# Autodesk Inventor assembly: Base
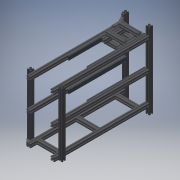
[picture p0: Inventor's stored thumbnail of the model, 180x180]
Saved by Autodesk Inventor 2016 (Build 200138000, 138)
## iProperties
Created: 2016-11-24
Part Number: Base
Material: 一般
Document SubType Name: Assembly
Designer: Daisuke
Author: Daisuke
## Documents named in this file (10)
- C:\Users\Daisuke\Documents\GitHub\CAD\Tomoato2016\Base\Base.iam
- C:\Users\Daisuke\Documents\GitHub\CAD\Tomoato2016\Base\HFS6-3030-750.ipt
- C:\Users\Daisuke\Documents\GitHub\CAD\Tomoato2016\Base\HFS6-3030-600.ipt
- C:\Users\Daisuke\Documents\GitHub\CAD\Tomoato2016\Base\HBLTF6-C_.ipt
- C:\Users\Daisuke\Documents\GitHub\CAD\Tomoato2016\Base\HFS6-3030-159.ipt
- C:\Users\Daisuke\Documents\GitHub\CAD\Tomoato2016\Base\HFS6-3030-500.ipt
- C:\Users\Daisuke\Documents\GitHub\CAD\Tomoato2016\Base\HBLFSNE6_.ipt
- C:\Users\Daisuke\Documents\GitHub\CAD\Tomoato2016\Base\SSRN3618.iam
- C:\Users\Daisuke\Documents\GitHub\CAD\Tomoato2016\Base\HFS6-3030-200.ipt
- C:\Users\Daisuke\Documents\GitHub\CAD\Tomoato2016\Base\HFS6-3030-140.ipt
## Components (26 placed, 9 different names)
1. HFS6-3030-750:1 — メイト:8, フラッシュ:9, フラッシュ:10, フラッシュ:32, フラッシュ:33, メイト:22, メイト:23
2. HFS6-3030-750:2 — メイト:9, フラッシュ:11, フラッシュ:12, メイト:21, メイト:24
3. HFS6-3030-750:3 — メイト:10, フラッシュ:13, フラッシュ:14, メイト:11, フラッシュ:16, フラッシュ:18, メイト:13, フラッシュ:19, フラッシュ:20, メイト:14, フラッシュ:23, フラッシュ:24, メイト:18, フラッシュ:28, フラッシュ:29
4. HFS6-3030-750:4 — メイト:7, フラッシュ:7, フラッシュ:8, メイト:12, フラッシュ:15, フラッシュ:17, フラッシュ:21, フラッシュ:22, メイト:15, フラッシュ:25, メイト:16, フラッシュ:26, フラッシュ:27
5. HFS6-3030-750:5 — メイト:6, フラッシュ:5, フラッシュ:6, フラッシュ:30, メイト:19, メイト:25
6. HFS6-3030-750:6 — メイト:1, フラッシュ:1, メイト:3, メイト:4, フラッシュ:31, メイト:20, メイト:26
7. HFS6-3030-600:1 — メイト:8, フラッシュ:9, フラッシュ:10, メイト:9, フラッシュ:11, フラッシュ:12, メイト:10, フラッシュ:13, フラッシュ:14
8. HFS6-3030-600:2 — メイト:1, フラッシュ:1, メイト:2, フラッシュ:2, フラッシュ:3, メイト:5, フラッシュ:4, メイト:6, フラッシュ:5, フラッシュ:6, メイト:7, フラッシュ:7, フラッシュ:8
9. HBLTF6-C_:1 — メイト:2, フラッシュ:2, フラッシュ:3, メイト:3
10. HBLTF6-C_:2 — メイト:4, メイト:5, フラッシュ:4
11. HFS6-3030-159:1 — メイト:14, フラッシュ:23, フラッシュ:24
12. HFS6-3030-159:2 — メイト:11, メイト:12, フラッシュ:15, フラッシュ:16, フラッシュ:17, フラッシュ:18
13. HFS6-3030-159:3 — メイト:13, フラッシュ:19, フラッシュ:20, フラッシュ:21, フラッシュ:22
14. HFS6-3030-500:1 — メイト:18, フラッシュ:28, フラッシュ:29
15. HFS6-3030-500:2 — メイト:15, フラッシュ:25, メイト:17
16. HBLFSNE6_:1 — メイト:16, メイト:17, フラッシュ:26, フラッシュ:27
17. SSRN3618:1 [sub-assembly] — フラッシュ:32, メイト:21, メイト:24
18. SSRN3618:2 [sub-assembly] — フラッシュ:31, メイト:20, メイト:26, フラッシュ:35, メイト:29, メイト:30
19. SSRN3618:3 [sub-assembly] — フラッシュ:33, メイト:22, メイト:23, フラッシュ:34, メイト:27, メイト:28
20. SSRN3618:4 [sub-assembly] — フラッシュ:30, メイト:19, メイト:25
21. HFS6-3030-200:1 — フラッシュ:34, メイト:27, メイト:28, フラッシュ:38, メイト:32, メイト:33, フラッシュ:39, フラッシュ:40, メイト:35, フラッシュ:43, フラッシュ:44
22. HFS6-3030-200:2 — フラッシュ:35, メイト:29, メイト:30, メイト:31, フラッシュ:36, フラッシュ:37, メイト:34, フラッシュ:41, フラッシュ:42
23. HFS6-3030-140:1 — メイト:31, フラッシュ:36, フラッシュ:37, フラッシュ:38, メイト:32
24. HFS6-3030-140:2 — メイト:33, フラッシュ:39, フラッシュ:40
25. HFS6-3030-140:3 — メイト:35, フラッシュ:41, フラッシュ:42
26. HFS6-3030-140:4 — メイト:34, フラッシュ:43, フラッシュ:44
## Relationships (79: Flush 44, Mate 35)
- メイト:1 [Mate]: HFS6-3030-750:6 ↔ HFS6-3030-600:2
- フラッシュ:1 [Flush]: HFS6-3030-750:6 ↔ HFS6-3030-600:2
- メイト:2 [Mate]: HFS6-3030-600:2 ↔ HBLTF6-C_:1
- フラッシュ:2 [Flush]: HFS6-3030-600:2 ↔ HBLTF6-C_:1
- フラッシュ:3 [Flush] (-5 mm): HFS6-3030-600:2 ↔ HBLTF6-C_:1
- メイト:3 [Mate]: HFS6-3030-750:6 ↔ HBLTF6-C_:1
- メイト:4 [Mate]: HFS6-3030-750:6 ↔ HBLTF6-C_:2
- メイト:5 [Mate]: HFS6-3030-600:2 ↔ HBLTF6-C_:2
- フラッシュ:4 [Flush] (5 mm): HFS6-3030-600:2 ↔ HBLTF6-C_:2
- メイト:6 [Mate]: HFS6-3030-750:5 ↔ HFS6-3030-600:2
- フラッシュ:5 [Flush]: HFS6-3030-750:5 ↔ HFS6-3030-600:2
- フラッシュ:6 [Flush] (285 mm): HFS6-3030-750:5 ↔ HFS6-3030-600:2
- メイト:7 [Mate]: HFS6-3030-750:4 ↔ HFS6-3030-600:2
- フラッシュ:7 [Flush]: HFS6-3030-750:4 ↔ HFS6-3030-600:2
- フラッシュ:8 [Flush] (55 mm): HFS6-3030-750:4 ↔ HFS6-3030-600:2
- メイト:8 [Mate]: HFS6-3030-750:1 ↔ HFS6-3030-600:1
- フラッシュ:9 [Flush]: HFS6-3030-750:1 ↔ HFS6-3030-600:1
- フラッシュ:10 [Flush] (55 mm): HFS6-3030-750:1 ↔ HFS6-3030-600:1
- メイト:9 [Mate]: HFS6-3030-750:2 ↔ HFS6-3030-600:1
- フラッシュ:11 [Flush]: HFS6-3030-750:2 ↔ HFS6-3030-600:1
- フラッシュ:12 [Flush] (285 mm): HFS6-3030-750:2 ↔ HFS6-3030-600:1
- メイト:10 [Mate]: HFS6-3030-750:3 ↔ HFS6-3030-600:1
- フラッシュ:13 [Flush]: HFS6-3030-750:3 ↔ HFS6-3030-600:1
- フラッシュ:14 [Flush] (55 mm): HFS6-3030-750:3 ↔ HFS6-3030-600:1
- メイト:11 [Mate]: HFS6-3030-750:3 ↔ HFS6-3030-159:2
- メイト:12 [Mate]: HFS6-3030-750:4 ↔ HFS6-3030-159:2
- フラッシュ:15 [Flush]: HFS6-3030-750:4 ↔ HFS6-3030-159:2
- フラッシュ:16 [Flush]: HFS6-3030-750:3 ↔ HFS6-3030-159:2
- フラッシュ:17 [Flush] (51 mm): HFS6-3030-750:4 ↔ HFS6-3030-159:2
- フラッシュ:18 [Flush] (51 mm): HFS6-3030-750:3 ↔ HFS6-3030-159:2
- メイト:13 [Mate]: HFS6-3030-750:3 ↔ HFS6-3030-159:3
- フラッシュ:19 [Flush]: HFS6-3030-750:3 ↔ HFS6-3030-159:3
- フラッシュ:20 [Flush] (51 mm): HFS6-3030-750:3 ↔ HFS6-3030-159:3
- フラッシュ:21 [Flush]: HFS6-3030-750:4 ↔ HFS6-3030-159:3
- フラッシュ:22 [Flush] (51 mm): HFS6-3030-750:4 ↔ HFS6-3030-159:3
- メイト:14 [Mate]: HFS6-3030-750:3 ↔ HFS6-3030-159:1
- フラッシュ:23 [Flush]: HFS6-3030-750:3 ↔ HFS6-3030-159:1
- フラッシュ:24 [Flush] (360 mm): HFS6-3030-750:3 ↔ HFS6-3030-159:1
- メイト:15 [Mate]: HFS6-3030-750:4 ↔ HFS6-3030-500:2
- フラッシュ:25 [Flush]: HFS6-3030-750:4 ↔ HFS6-3030-500:2
- メイト:16 [Mate]: HFS6-3030-750:4 ↔ HBLFSNE6_:1
- メイト:17 [Mate]: HFS6-3030-500:2 ↔ HBLFSNE6_:1
- フラッシュ:26 [Flush]: HFS6-3030-750:4 ↔ HBLFSNE6_:1
- フラッシュ:27 [Flush] (5 mm): HFS6-3030-750:4 ↔ HBLFSNE6_:1
- メイト:18 [Mate]: HFS6-3030-750:3 ↔ HFS6-3030-500:1
- フラッシュ:28 [Flush]: HFS6-3030-750:3 ↔ HFS6-3030-500:1
- フラッシュ:29 [Flush] (-30 mm): HFS6-3030-750:3 ↔ HFS6-3030-500:1
- フラッシュ:30 [Flush]: HFS6-3030-750:5 ↔ SSRN3618:4
- メイト:19 [Mate]: HFS6-3030-750:5 ↔ SSRN3618:4
- フラッシュ:31 [Flush]: HFS6-3030-750:6 ↔ SSRN3618:2
- メイト:20 [Mate]: HFS6-3030-750:6 ↔ SSRN3618:2
- フラッシュ:32 [Flush]: HFS6-3030-750:1 ↔ SSRN3618:1
- メイト:21 [Mate]: HFS6-3030-750:2 ↔ SSRN3618:1
- フラッシュ:33 [Flush]: HFS6-3030-750:1 ↔ SSRN3618:3
- メイト:22 [Mate]: HFS6-3030-750:1 ↔ SSRN3618:3
- メイト:23 [Mate]: HFS6-3030-750:1 ↔ SSRN3618:3
- メイト:24 [Mate]: HFS6-3030-750:2 ↔ SSRN3618:1
- メイト:25 [Mate]: HFS6-3030-750:5 ↔ SSRN3618:4
- メイト:26 [Mate]: HFS6-3030-750:6 ↔ SSRN3618:2
- フラッシュ:34 [Flush]: SSRN3618:3 ↔ HFS6-3030-200:1
- メイト:27 [Mate]: SSRN3618:3 ↔ HFS6-3030-200:1
- メイト:28 [Mate]: SSRN3618:3 ↔ HFS6-3030-200:1
- フラッシュ:35 [Flush]: SSRN3618:2 ↔ HFS6-3030-200:2
- メイト:29 [Mate]: SSRN3618:2 ↔ HFS6-3030-200:2
- メイト:30 [Mate]: SSRN3618:2 ↔ HFS6-3030-200:2
- メイト:31 [Mate]: HFS6-3030-200:2 ↔ HFS6-3030-140:1
- フラッシュ:36 [Flush]: HFS6-3030-200:2 ↔ HFS6-3030-140:1
- フラッシュ:37 [Flush] (-30 mm): HFS6-3030-200:2 ↔ HFS6-3030-140:1
- フラッシュ:38 [Flush] (30 mm): HFS6-3030-200:1 ↔ HFS6-3030-140:1
- メイト:32 [Mate]: HFS6-3030-200:1 ↔ HFS6-3030-140:1
- メイト:33 [Mate]: HFS6-3030-200:1 ↔ HFS6-3030-140:2
- フラッシュ:39 [Flush]: HFS6-3030-200:1 ↔ HFS6-3030-140:2
- フラッシュ:40 [Flush] (30 mm): HFS6-3030-200:1 ↔ HFS6-3030-140:2
- メイト:34 [Mate]: HFS6-3030-200:2 ↔ HFS6-3030-140:4
- メイト:35 [Mate]: HFS6-3030-200:1 ↔ HFS6-3030-140:3
- フラッシュ:41 [Flush]: HFS6-3030-200:2 ↔ HFS6-3030-140:3
- フラッシュ:42 [Flush] (30 mm): HFS6-3030-200:2 ↔ HFS6-3030-140:3
- フラッシュ:43 [Flush]: HFS6-3030-200:1 ↔ HFS6-3030-140:4
- フラッシュ:44 [Flush] (30 mm): HFS6-3030-200:1 ↔ HFS6-3030-140:4
